# Autodesk Inventor assembly: Matriz centelladora 15X14
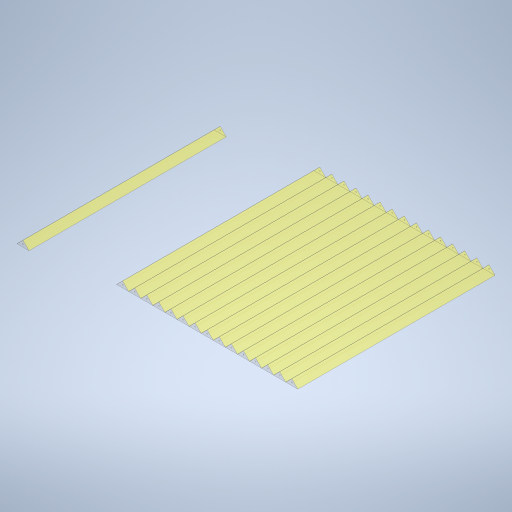
[picture p0: Inventor's stored thumbnail of the model, 512x512]
Saved by Autodesk Inventor 2024.2 (Build 282272000, 272)
## iProperties
Created: 2024-08-22
Part Number: Matriz centelladora 15X14
Document SubType Name: Assembly
Designer: ja.restrepo1
Author: ja.restrepo1
## Documents named in this file (2)
- I:\MICROMECANICA\ALTAS ENERGIAS\Deteccion de Muones\Detectores\Detectores centelladores\Partes Detectores centelladores\PARTES DC\Centelladora CD\Matriz centelladora 15X14.iam
- I:\MICROMECANICA\ALTAS ENERGIAS\Deteccion de Muones\Detectores\Detectores centelladores\Partes Detectores centelladores\PARTES DC\Centelladora CD\Centelladora triangular.ipt
## Components (16 placed, 1 different names)
1. Centelladora triangular:2
2. Centelladora triangular:1 — Flush:1, Flush:2, Flush:3, Mate:1
3. Centelladora triangular:3
4. Centelladora triangular:4
5. Centelladora triangular:5
6. Centelladora triangular:6
7. Centelladora triangular:7
8. Centelladora triangular:8
9. Centelladora triangular:9
10. Centelladora triangular:10
11. Centelladora triangular:11
12. Centelladora triangular:12
13. Centelladora triangular:13
14. Centelladora triangular:14
15. Centelladora triangular:15
16. Centelladora triangular:16
## Component patterns: Matriz 15 (15 elements)
## Relationships (4: Flush 3, Mate 1)
- Flush:1: Centelladora triangular:1
- Flush:2: Centelladora triangular:1
- Flush:3: Centelladora triangular:1
- Mate:1: Centelladora triangular:1
